# Autodesk Inventor assembly: Body_Prototype1
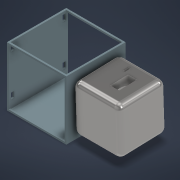
[picture p0: Inventor's stored thumbnail of the model, 180x180]
Saved by Autodesk Inventor 2021 (Build 250183000, 183)
## iProperties
Created: 2022-02-15
Part Number: Body_Prototype1
Document SubType Name: Assembly
Designer: utkaa
Author: utkaa
## Documents named in this file (3)
- C:\Users\utkaa\OneDrive\Desktop\OneDrive-2020-09-15\Robocon\Body_Prototype1.iam
- C:\Users\utkaa\OneDrive\Desktop\OneDrive-2020-09-15\Robocon\Body_prototype2.ipt
- C:\Users\utkaa\OneDrive\Desktop\OneDrive-2020-09-15\Robocon\Head_prototype2.ipt
## Components (2 placed, 2 different names)
1. Body_prototype2:1 — Mate:1, Mate:2
2. Head_prototype2:1 — Mate:1, Mate:2
## Relationships (4: Mate 2, Symmetry 2)
- Mate:1: Body_prototype2:1 ↔ Head_prototype2:1
- Mate:2: Body_prototype2:1 ↔ Head_prototype2:1
- Symmetry:1
- Symmetry:2
